# Autodesk Inventor assembly: 2inTurret
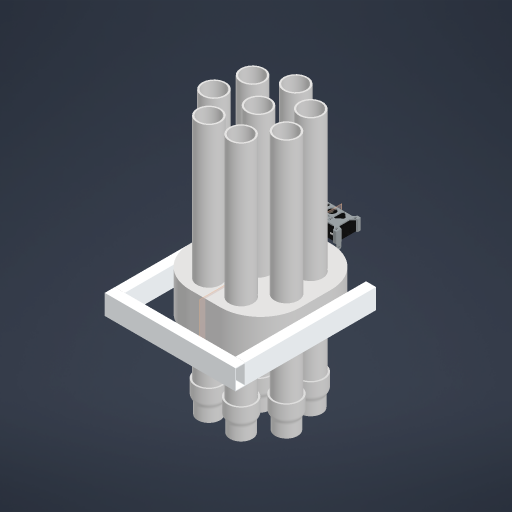
[picture p0: Inventor's stored thumbnail of the model, 512x512]
Saved by Autodesk Inventor 2023 (Build 270158000, 158)
## iProperties
Created: 2022-06-22
Part Number: 2inTurret
Document SubType Name: Assembly
Designer: timmy
Author: timmy
## Documents named in this file (4)
- R:\Inventor\RoboCatz\T-Shirt\Rev2-Better\2inTurret.iam
- R:\Inventor\RoboCatz\T-Shirt\Rev2-Better\2inShooters.iam
- R:\Inventor\RoboCatz\T-Shirt\Rev2-Better\am-3214 2x1x0625 wall tubing.ipt
- R:\Inventor\RoboCatz\T-Shirt\Rev2-Better\Limelight.iam
## Components (5 placed, 3 different names)
1. 2inShooters:1 [sub-assembly] — Mate:1, Mate:2, Mate:3, Mate:4, Angle:1, Flush:7, Angle:2
2. am-3214 2x1x0625 wall tubing:1 — Mate:1, Mate:2, Flush:1, Mate:5, Flush:2, Flush:3
3. am-3214 2x1x0625 wall tubing:2 — Mate:3, Mate:4, Flush:1, Angle:1
4. am-3214 2x1x0625 wall tubing:3 — Mate:5, Flush:2, Flush:3
5. Limelight:1 [sub-assembly] — Flush:7, Angle:2
## Relationships (11: Mate 5, Flush 4, Angle 2)
- Mate:1: 2inShooters:1 ↔ am-3214 2x1x0625 wall tubing:1
- Mate:2: 2inShooters:1 ↔ am-3214 2x1x0625 wall tubing:1
- Mate:3: 2inShooters:1 ↔ am-3214 2x1x0625 wall tubing:2
- Mate:4: 2inShooters:1 ↔ am-3214 2x1x0625 wall tubing:2
- Flush:1: am-3214 2x1x0625 wall tubing:1 ↔ am-3214 2x1x0625 wall tubing:2
- Mate:5: am-3214 2x1x0625 wall tubing:1 ↔ am-3214 2x1x0625 wall tubing:3
- Flush:2: am-3214 2x1x0625 wall tubing:1 ↔ am-3214 2x1x0625 wall tubing:3
- Flush:3: am-3214 2x1x0625 wall tubing:1 ↔ am-3214 2x1x0625 wall tubing:3
- Angle:1 (0 deg): 2inShooters:1 ↔ am-3214 2x1x0625 wall tubing:2
- Flush:7: 2inShooters:1 ↔ Limelight:1
- Angle:2 (180 deg): 2inShooters:1 ↔ Limelight:1
